# Autodesk Inventor assembly: FULL SWERVE DRIVE ASSEMBLY!  2!
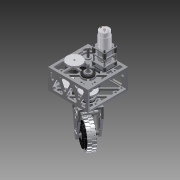
[picture p0: Inventor's stored thumbnail of the model, 180x180]
Saved by Autodesk Inventor 2012 (Build 160160000, 160)
## iProperties
Created: 2013-01-01
Part Number: FULL SWERVE DRIVE ASSEMBLY!  2!
Document SubType Name: Assembly
Designer: Bryce
Author: Bryce
## Documents named in this file (11)
- C:\Users\Bryce\Dropbox\Inventor Design Project Files\Independent Swerves\Inventor 2012\FULL SWERVE DRIVE ASSEMBLY!  2! (Bryce Croucher's conflicted copy 2013-01-15).iam
- C:\Users\Bryce\Dropbox\Inventor Design Project Files\Independent Swerves\Inventor 2012\upper gearbox frame.ipt
- C:\Users\Bryce\Dropbox\Inventor Design Project Files\Independent Swerves\Inventor 2012\collar bearing systom.ipt
- C:\Users\Bryce\Dropbox\Inventor Design Project Files\Independent Swerves\Inventor 2012\Lower box main assembly 2.iam
- C:\Users\Bryce\Dropbox\Inventor Design Project Files\Independent Swerves\Imported Components\BD Gearbox and Bracket Assy 3.iam
- C:\Users\Bryce\Dropbox\Inventor Design Project Files\Independent Swerves\Imported Components\CIM Motor.iam
- C:\Users\Bryce\Dropbox\Inventor Design Project Files\Independent Swerves\Inventor 2012\turn encoder assembly.iam
- C:\Users\Bryce\Dropbox\Inventor Design Project Files\Independent Swerves\Imported Components\Imported Components\48-5m09-6a5\48-5m09-6a5.ipt
- C:\Users\Bryce\Dropbox\Inventor Design Project Files\Independent Swerves\Inventor 2012\frame assembly 2.iam
- C:\Users\Bryce\Dropbox\Inventor Design Project Files\Independent Swerves\Inventor 2012\frame assembly 3.iam
- C:\Users\Bryce\Dropbox\Inventor Design Project Files\Independent Swerves\Imported Components\encoder gear turn.ipt
## Components (12 placed, 10 different names)
1. upper gearbox frame:1 — Mate:1, Mate:2, Mate:3, Mate:4, Mate:6, Mate:7, Mate:8, Mate:9, Mate:11, Mate:16, Mate:17, Mate:18, Mate:20, Mate:21, Mate:22, Angle:2, Mate:24, Mate:25, Mate:26, Mate:27, Flush:5, Flush:6, Mate:29
2. collar bearing systom:1 — Mate:1, Mate:2, Flush:1
3. collar bearing systom:2 — Mate:3, Mate:4, Mate:5
4. Lower box main assembly 2:1 [sub-assembly] — Mate:5, Flush:1, Flush:4, Mate:28, Flush:7
5. BD Gearbox and Bracket Assy 3:1 [sub-assembly] — Mate:6, Mate:7, Mate:8, Mate:9
6. CIM Motor:1 [sub-assembly] — Mate:11, Mate:20, Mate:21, Mate:22
7. turn encoder assembly:1 [sub-assembly] — Mate:17, Mate:18, Angle:1, Angle:2, Rotation:1
8. turn encoder assembly:2 [sub-assembly] — Mate:16, Angle:1, Mate:29
9. encoder gear turn:1 — Mate:28, Flush:7, Rotation:1
10. 48-5m09-6a5:1 — Flush:4
11. frame assembly 2:1 [sub-assembly] — Mate:24, Mate:25, Mate:26
12. frame assembly 3:1 [sub-assembly] — Mate:27, Flush:5, Flush:6
## Relationships (31: Mate 22, Flush 6, Angle 2, RelateRotation 1)
- Mate:1: upper gearbox frame:1 ↔ collar bearing systom:1
- Mate:2: upper gearbox frame:1 ↔ collar bearing systom:1
- Mate:3: upper gearbox frame:1 ↔ collar bearing systom:2
- Mate:4: upper gearbox frame:1 ↔ collar bearing systom:2
- Mate:5: collar bearing systom:2 ↔ Lower box main assembly 2:1
- Flush:1 (-1.27 mm): collar bearing systom:1 ↔ Lower box main assembly 2:1
- Mate:6: upper gearbox frame:1 ↔ BD Gearbox and Bracket Assy 3:1
- Mate:7 (6.35 mm): upper gearbox frame:1 ↔ BD Gearbox and Bracket Assy 3:1
- Mate:8 (6.35 mm): upper gearbox frame:1 ↔ BD Gearbox and Bracket Assy 3:1
- Mate:9 (6.35 mm): upper gearbox frame:1 ↔ BD Gearbox and Bracket Assy 3:1
- Mate:11: upper gearbox frame:1 ↔ CIM Motor:1
- Mate:16: upper gearbox frame:1 ↔ turn encoder assembly:2
- Mate:17: upper gearbox frame:1 ↔ turn encoder assembly:1
- Mate:18: upper gearbox frame:1 ↔ turn encoder assembly:1
- [Flush]: turn encoder assembly:1 ↔ encoder gear turn:1
- Mate:20 (3.175 mm): upper gearbox frame:1 ↔ CIM Motor:1
- Mate:21 (9.525 mm): upper gearbox frame:1 ↔ CIM Motor:1
- Mate:22 (9.525 mm): upper gearbox frame:1 ↔ CIM Motor:1
- Flush:4: Lower box main assembly 2:1 ↔ 48-5m09-6a5:1
- Angle:1 (0 deg): turn encoder assembly:1 ↔ turn encoder assembly:2
- Angle:2 (180 deg): upper gearbox frame:1 ↔ turn encoder assembly:1
- Mate:24: upper gearbox frame:1 ↔ frame assembly 2:1
- Mate:25: upper gearbox frame:1 ↔ frame assembly 2:1
- Mate:26: upper gearbox frame:1 ↔ frame assembly 2:1
- Mate:27: upper gearbox frame:1 ↔ frame assembly 3:1
- Flush:5: upper gearbox frame:1 ↔ frame assembly 3:1
- Flush:6: upper gearbox frame:1 ↔ frame assembly 3:1
- Mate:28: Lower box main assembly 2:1 ↔ encoder gear turn:1
- Flush:7: Lower box main assembly 2:1 ↔ encoder gear turn:1
- Rotation:1 [RelateRotation] (1 ul): turn encoder assembly:1 ↔ encoder gear turn:1
- Mate:29: upper gearbox frame:1 ↔ turn encoder assembly:2
